# Autodesk Inventor assembly: Shooter Assembly v2 (copy)
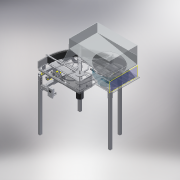
[picture p0: Inventor's stored thumbnail of the model, 180x180]
Saved by Autodesk Inventor 2013 (Build 170138000, 138)
## iProperties
Created: 2013-01-15
Part Number: Shooter Assembly v2 (copy)
Document SubType Name: Assembly
Designer: actoennies
Mass: 9112.82 g
Surface Area: 29351.4 cm^2
Volume: 4689.84 cm^3
Density: 1.9431 g/cm^3
Author: actoennies
## Documents named in this file (49)
- C:\Users\Arpan\Documents\GitHub\frc2013CAD\Launcher\Shooter\Shooter Assembly v2 (copy).iam
- C:\Users\Arpan\Documents\GitHub\frc2013CAD\Launcher\Shooter\Bearing Mount v1.ipt
- C:\Users\Arpan\Documents\GitHub\frc2013CAD\Launcher\Shooter\Outer Rail v1.ipt
- C:\Users\Arpan\Documents\GitHub\frc2013CAD\Launcher\Shooter\Runner Rails v2.ipt
- C:\Users\Arpan\Documents\GitHub\frc2013CAD\Launcher\Shooter\Bearing.ipt
- C:\Users\Arpan\Documents\GitHub\frc2013CAD\Launcher\Shooter\Shooter Mounter.ipt
- C:\Users\Arpan\Documents\GitHub\frc2013CAD\Launcher\Shooter\Bearing Mount 2 v1.ipt
- C:\Users\Arpan\Documents\GitHub\frc2013CAD\Launcher\Shooter\Shorter Shaft.ipt
- C:\Users\Arpan\Documents\GitHub\frc2013CAD\Launcher\Shooter\Spacer Rube.ipt
- C:\Users\Arpan\Documents\GitHub\frc2013CAD\Launcher\Shooter\Edge Mount.ipt
- C:\Users\Arpan\Documents\GitHub\frc2013CAD\Launcher\Shooter\Square Tube.ipt
- C:\Users\Arpan\Documents\GitHub\frc2013CAD\Launcher\Shooter\Flange Bearing Mount Tower.ipt
- C:\Users\Arpan\Documents\GitHub\frc2013CAD\Launcher\Shooter\Flange Bearing Mount Tower Mirror.ipt
- C:\Users\Arpan\Documents\GitHub\frc2013CAD\Launcher\Shooter\Bearing Mount Top.ipt
- C:\Users\Arpan\Documents\GitHub\frc2013CAD\Launcher\Shooter\Square Motor Mount.ipt
- C:\Users\Arpan\Documents\GitHub\frc2013CAD\Launcher\Shooter\Shooter Assembly v2\Design Accelerator\Spur Gears1.iam
- C:\Users\Arpan\Documents\GitHub\frc2013CAD\Launcher\Parts\Imported Components\Snow Blower Motor\Snow Blower Motor.iam
- C:\Users\Arpan\Documents\GitHub\frc2013CAD\Launcher\Shooter\Snowblower Motor Mount.ipt
- C:\Users\Arpan\Documents\GitHub\frc2013CAD\Launcher\Shooter\8mm shaft.ipt
- C:\Users\Arpan\Documents\GitHub\frc2013CAD\Launcher\Shooter\CIM Bearing.ipt
- C:\Users\Arpan\Documents\GitHub\frc2013CAD\Launcher\Shooter\Square Tube 2.ipt
- C:\Users\Arpan\Documents\GitHub\frc2013CAD\Launcher\Parts\CIM Motor\Motors_FR801-001.iam
- C:\Users\Arpan\Documents\GitHub\frc2013CAD\Launcher\Shooter\Cim Mount.ipt
- C:\Users\Arpan\Documents\GitHub\frc2013CAD\Launcher\Shooter\Camera Traffic Light Mount.ipt
- C:\Users\Arpan\Documents\GitHub\frc2013CAD\Launcher\Shooter\Square Tube 3.ipt
- C:\Users\Arpan\Documents\GitHub\frc2013CAD\Launcher\Shooter\edge mount shortened.ipt
- C:\Users\Arpan\Documents\GitHub\frc2013CAD\Launcher\Shooter\Camera.ipt
- C:\Users\Arpan\Documents\GitHub\frc2013CAD\Launcher\Shooter\Square Tube 6.ipt
- C:\Users\Arpan\Documents\GitHub\frc2013CAD\Launcher\Parts\NR-025_5-D(F,D-770).iam
- C:\Users\Arpan\Documents\GitHub\frc2013CAD\Launcher\Parts\Imported Components\E3-X-315-X-D-3-X\E3-X-315-X-D-3-X.ipt
- C:\Users\Arpan\Documents\GitHub\frc2013CAD\Launcher\Shooter\Gusset.ipt
- C:\Users\Arpan\Documents\GitHub\frc2013CAD\Launcher\Shooter\Gusset 2.ipt
- C:\Users\Arpan\Documents\GitHub\frc2013CAD\Launcher\Shooter\Gusset 3.ipt
- C:\Users\Arpan\Documents\GitHub\frc2013CAD\Launcher\Shooter\Gusset 4.ipt
- C:\Users\Arpan\Documents\GitHub\frc2013CAD\Launcher\Shooter\Inner Mount.ipt
- C:\Users\Arpan\Documents\GitHub\frc2013CAD\Launcher\Shooter\Gusset 5.ipt
- C:\Users\Arpan\Documents\GitHub\frc2013CAD\Launcher\Shooter\Hard Stop.ipt
- C:\Users\Arpan\Documents\GitHub\frc2013CAD\Launcher\Shooter\Gusset Connector 2.ipt
- C:\Users\Arpan\Documents\GitHub\frc2013CAD\Launcher\Shooter\L-Channel Strenght.ipt
- C:\Users\Arpan\Documents\GitHub\frc2013CAD\Launcher\Shooter\Gear for Angle.ipt
- C:\Users\Arpan\Documents\GitHub\frc2013CAD\Launcher\Shooter\Encoder Mount 2.ipt
- \\NNHSSRV2.hs.sd203.org\ACToennies$\Robotics\Shooter\Gear Plate.ipt
- \\NNHSSRV2.hs.sd203.org\ACToennies$\Robotics\Shooter\Gear Plate 2.ipt
- C:\Users\Arpan\Documents\GitHub\frc2013CAD\Launcher\Shooter\Wheel Shields.ipt
- C:\Users\Arpan\Documents\GitHub\frc2013CAD\Launcher\Shooter\Rubber Cushion.ipt
- \\NNHSSRV2.hs.sd203.org\ACToennies$\Inventor\Pneumatic Wheel.iam
- C:\Users\Arpan\Documents\GitHub\frc2013CAD\Launcher\Shooter\Puller Hook.ipt
- C:\Users\Arpan\Documents\GitHub\frc2013CAD\Launcher\Shooter\Bucketr.ipt
- C:\Users\Arpan\Documents\GitHub\frc2013CAD\Launcher\Shooter\Hopper.ipt
## Components (71 placed, 48 different names)
1. Bearing Mount v1:1 — Insert:13, Insert:26, Insert:27, Mate:62, Mate:63, Flush:70, Insert:60, Insert:61, Mate:167, Flush:128, Mate:255
2. Outer Rail v1:1 — Insert:13, Insert:48, Flush:70, Mate:252
3. Runner Rails v2:1 — Insert:60, Insert:61, Angle:16, Mate:257, Mate:258, Mate:259, Flush:130, Flush:131
4. Shooter Mounter:1 — Insert:26, Insert:27, Insert:34, Flush:11, Insert:35, Insert:36, Insert:37, Insert:38, Flush:19, Mate:45, Flush:40, Flush:64, Angle:6, Angle:8, Mate:226, Flush:114, Flush:115, Mate:229, Mate:230, Flush:116, Mate:232, Flush:117, Mate:238, Mate:246, Angle:15, Mate:247, Mate:248, Mate:249, Flush:124
5. Spacer Rube:1 — Insert:34, Flush:11
6. Bearing Mount 2 v1:1 — Insert:37, Insert:38, Insert:40
7. Bearing Mount 2 v1:2 — Insert:35, Insert:36, Insert:39
8. Bearing:3 — Insert:40, Flush:13, Mate:14, Mate:15
9. Bearing:4 — Insert:39, Mate:36, Mate:44
10. Shorter Shaft:2 — Flush:13, Mate:14, Mate:15, Mate:38
11. Edge Mount:2 — Flush:34, Mate:104, Flush:48, Mate:106, Flush:68, Mate:174, Flush:74, Mate:220, Mate:222
12. Square Tube:2 — Flush:19, Flush:23, Mate:52, Flush:27, Mate:81, Flush:32, Mate:125, Mate:126, Mate:130, Flush:50, Angle:8, Mate:192, Flush:83, Mate:217, Flush:103, Flush:112, Insert:71, Insert:72
13. Flange Bearing Mount Tower:1 — Insert:43, Flush:112, Flush:113
14. Bearing:5 — Insert:43, Mate:36
15. Flange Bearing Mount Tower Mirror:1 — Flush:55, Mate:135, Flush:111, Insert:70
16. Bearing:6 — Mate:38, Insert:70
17. Bearing Mount Top:1 — Insert:48, Mate:65, Mate:66, Mate:253, Tangent:1
18. Square Motor Mount:1 — Flush:23, Mate:47, Mate:51, Flush:27, Mate:131, Mate:197, Mate:198, Flush:86, Flush:96, Flush:106
19. Spur Gears:1 [sub-assembly] — Mate:44, Mate:45, Flush:25, Mate:46, Angle:2, Flush:64, Angle:6, Mate:227, Mate:228, Mate:231, Mate:233, Flush:120, Mate:239, Flush:122
20. Snow Blower Motor:1 [sub-assembly] — Flush:25, Mate:46, Angle:2, Insert:81, Insert:82, Mate:245
21. Snowblower Motor Mount:1 — Mate:47, Mate:51, Mate:52, Mate:240, Insert:76, Insert:78, Insert:79, Insert:81, Insert:82, Mate:241, Mate:242, Mate:243, Mate:244
22. 8mm shaft:1 — Mate:67, Mate:82, Mate:83, Mate:84, Mate:86, Mate:167, Mate:254
23. CIM Bearing:1 — Mate:65, Mate:66, Mate:67
24. CIM Bearing:2 — Mate:62, Mate:63
25. Square Tube 2:1 — Mate:81, Flush:32, Flush:34, Mate:106, Mate:124, Flush:49, Mate:126, Mate:173, Mate:186, Flush:80, Mate:193, Mate:216, Mate:219, Flush:104, Flush:111, Flush:113
26. Motors_FR801-001:1 [sub-assembly] — Mate:82, Mate:83, Mate:84, Mate:143, Mate:144, Mate:145
27. Cim Mount:1 — Flush:40, Mate:143, Mate:144, Mate:145
28. Camera Traffic Light Mount:1 — Mate:127, Mate:128, Mate:129, Insert:83, Insert:84
29. Square Tube 3:1 — Mate:104, Flush:48, Flush:55, Mate:135, Mate:173, Mate:174, Flush:74, Mate:175, Mate:187, Mate:206, Flush:90, Mate:221, Flush:105, Flush:110
30. edge mount shortened:1 — Mate:124, Mate:125, Flush:49, Mate:196, Flush:85, Mate:215, Flush:102, Mate:218, Mate:223, Flush:107
31. Camera:1 — Mate:127, Mate:128, Mate:129
32. Edge Mount:3 — Mate:130, Mate:131, Flush:50, Mate:199, Mate:209, Flush:97, Mate:212, Mate:260, Mate:261
33. Square Tube 6:1 — Mate:175, Flush:91, Mate:207, Flush:93, Mate:208, Flush:94, Flush:95, Flush:110, Mate:224, Insert:73, Insert:74
34. NR-025_5-D(F,D-770):1 [sub-assembly] — Mate:246, Angle:15, Mate:247, Mate:256, Flush:129
35. Gusset:3 — Mate:186, Flush:80, Mate:187
36. Gusset:4 — Mate:196, Mate:197, Flush:85
37. Gusset:5 — Mate:192, Mate:193, Flush:83
38. Gusset:8 — Mate:198, Mate:199, Flush:86
39. Gusset 2:1 — Mate:206, Flush:90, Flush:91
40. Gusset 3:2 — Mate:209, Flush:96, Flush:97
41. Gusset 3:3 — Mate:208, Flush:94, Flush:95, Flush:108
42. Gusset 3:4 — Mate:207, Flush:93, Mate:225
43. Gusset 4:1 — Mate:212, Mate:260, Mate:261, Insert:83, Insert:84
44. Gusset 4:2
45. Gusset 4:3 — Mate:217, Mate:218, Flush:103
46. Gusset 4:4 — Mate:215, Flush:102, Mate:216
47. Gusset 4:5 — Mate:219, Mate:220, Flush:104
48. Gusset 4:6 — Mate:221, Mate:222, Flush:105
49. Gusset 3:5 — Mate:223, Flush:106, Flush:107
50. Inner Mount:1 — Flush:108, Mate:224, Mate:225
51. Gusset 5:1 — Flush:115, Mate:228, Mate:229
52. Gusset 5:2 — Mate:226, Mate:227, Flush:114
53. Gusset 5:3 — Mate:230, Mate:231, Flush:116
54. Gusset 5:4 — Mate:232, Mate:233, Flush:117
55. Hard Stop:1 — Insert:71, Insert:72
56. Gusset Connector 2:1 — Insert:73, Insert:74
57. L-Channel Strenght:1 — Mate:238, Mate:248, Mate:249, Mate:250, Flush:125
58. Gear for Angle:1 — Flush:120, Mate:239, Mate:240, Flush:121
59. CIM Bearing:3 — Insert:76, Insert:77
60. 8mm shaft:2 — Insert:77, Flush:121
61. E3-X-315-X-D-3-X:2 — Insert:80, Angle:14
62. Encoder Mount 2:1 — Insert:78, Insert:79, Insert:80, Angle:14
63. Gear Plate:1 — Mate:241, Mate:242, Flush:122, Flush:123
64. Gear Plate 2:1 — Mate:243, Mate:244, Flush:123
65. Wheel Shields:1 — Mate:250, Flush:124, Flush:125, Mate:251, Flush:126, Flush:127
66. Wheel Shields:2 — Mate:251, Flush:126, Flush:127, Angle:17
67. Rubber Cushion:1 — Mate:252, Mate:253, Flush:128
68. Pneumatic Wheel:1 [sub-assembly] — Mate:254, Mate:255
69. Puller Hook:1 — Mate:256, Flush:129, Angle:16
70. Bucketr:1 — Mate:257, Tangent:1, Mate:258, Angle:17
71. Hopper:1 — Mate:259, Flush:130, Flush:131
## Relationships (185: Mate 94, Flush 55, Insert 28, Angle 7, Tangent 1)
- Insert:13: Bearing Mount v1:1 ↔ Outer Rail v1:1
- Insert:26: Bearing Mount v1:1 ↔ Shooter Mounter:1
- Insert:27: Bearing Mount v1:1 ↔ Shooter Mounter:1
- Insert:34: Shooter Mounter:1 ↔ Spacer Rube:1
- Flush:11: Shooter Mounter:1 ↔ Spacer Rube:1
- Insert:35: Shooter Mounter:1 ↔ Bearing Mount 2 v1:2
- Insert:36: Shooter Mounter:1 ↔ Bearing Mount 2 v1:2
- Insert:37: Shooter Mounter:1 ↔ Bearing Mount 2 v1:1
- Insert:38: Shooter Mounter:1 ↔ Bearing Mount 2 v1:1
- Insert:39: Bearing Mount 2 v1:2 ↔ Bearing:4
- Insert:40: Bearing Mount 2 v1:1 ↔ Bearing:3
- Flush:13 (-25.4 mm): Bearing:3 ↔ Shorter Shaft:2
- Mate:14: Bearing:3 ↔ Shorter Shaft:2
- Mate:15: Bearing:3 ↔ Shorter Shaft:2
- Insert:43: Flange Bearing Mount Tower:1 ↔ Bearing:5
- Flush:19: Shooter Mounter:1 ↔ Square Tube:2
- Mate:36: Bearing:4 ↔ Bearing:5
- Mate:38: Shorter Shaft:2 ↔ Bearing:6
- Insert:48 (12.7 mm): Outer Rail v1:1 ↔ Bearing Mount Top:1
- Flush:23 (152.4 mm): Square Tube:2 ↔ Square Motor Mount:1
- Mate:44: Bearing:4 ↔ Spur Gears:1
- Mate:45 (25.4 mm): Shooter Mounter:1 ↔ Spur Gears:1
- Flush:25 (-3.175 mm): Spur Gears:1 ↔ Snow Blower Motor:1
- Mate:46: Spur Gears:1 ↔ Snow Blower Motor:1
- Angle:2 (0 deg): Spur Gears:1 ↔ Snow Blower Motor:1
- Mate:47: Square Motor Mount:1 ↔ Snowblower Motor Mount:1
- Mate:51: Square Motor Mount:1 ↔ Snowblower Motor Mount:1
- Mate:52: Square Tube:2 ↔ Snowblower Motor Mount:1
- Flush:27: Square Tube:2 ↔ Square Motor Mount:1
- Mate:62: Bearing Mount v1:1 ↔ CIM Bearing:2
- Mate:63: Bearing Mount v1:1 ↔ CIM Bearing:2
- Mate:65: Bearing Mount Top:1 ↔ CIM Bearing:1
- Mate:66: Bearing Mount Top:1 ↔ CIM Bearing:1
- Mate:67: 8mm shaft:1 ↔ CIM Bearing:1
- Mate:81: Square Tube:2 ↔ Square Tube 2:1
- Flush:32: Square Tube:2 ↔ Square Tube 2:1
- Flush:34: Edge Mount:2 ↔ Square Tube 2:1
- Mate:82: 8mm shaft:1 ↔ Motors_FR801-001:1
- Mate:83: 8mm shaft:1 ↔ Motors_FR801-001:1
- Mate:84: 8mm shaft:1 ↔ Motors_FR801-001:1
- Mate:86: 8mm shaft:1
- Flush:40: Shooter Mounter:1 ↔ Cim Mount:1
- Mate:104: Edge Mount:2 ↔ Square Tube 3:1
- Flush:48: Edge Mount:2 ↔ Square Tube 3:1
- Mate:106: Edge Mount:2 ↔ Square Tube 2:1
- Mate:124: Square Tube 2:1 ↔ edge mount shortened:1
- Mate:125: Square Tube:2 ↔ edge mount shortened:1
- Flush:49: Square Tube 2:1 ↔ edge mount shortened:1
- Mate:126: Square Tube:2 ↔ Square Tube 2:1
- Mate:127: Camera Traffic Light Mount:1 ↔ Camera:1
- Mate:128: Camera Traffic Light Mount:1 ↔ Camera:1
- Mate:129: Camera Traffic Light Mount:1 ↔ Camera:1
- Mate:130: Square Tube:2 ↔ Edge Mount:3
- Mate:131: Square Motor Mount:1 ↔ Edge Mount:3
- Flush:50: Square Tube:2 ↔ Edge Mount:3
- Flush:55: Flange Bearing Mount Tower Mirror:1 ↔ Square Tube 3:1
- Mate:135: Flange Bearing Mount Tower Mirror:1 ↔ Square Tube 3:1
- Mate:143: Motors_FR801-001:1 ↔ Cim Mount:1
- Mate:144: Motors_FR801-001:1 ↔ Cim Mount:1
- Mate:145: Motors_FR801-001:1 ↔ Cim Mount:1
- Flush:64 (3.175 mm): Shooter Mounter:1 ↔ Spur Gears:1
- Flush:68 (-950.9125 mm): Edge Mount:2
- Flush:70: Bearing Mount v1:1 ↔ Outer Rail v1:1
- Insert:60: Bearing Mount v1:1 ↔ Runner Rails v2:1
- Insert:61: Bearing Mount v1:1 ↔ Runner Rails v2:1
- Angle:6 (180 deg): Shooter Mounter:1 ↔ Spur Gears:1
- Mate:167: Bearing Mount v1:1 ↔ 8mm shaft:1
- Angle:8 (180 deg): Shooter Mounter:1 ↔ Square Tube:2
- Mate:173: Square Tube 2:1 ↔ Square Tube 3:1
- Mate:174: Edge Mount:2 ↔ Square Tube 3:1
- Flush:74: Edge Mount:2 ↔ Square Tube 3:1
- Mate:175: Square Tube 3:1 ↔ Square Tube 6:1
- Mate:186: Square Tube 2:1 ↔ Gusset:3
- Flush:80: Square Tube 2:1 ↔ Gusset:3
- Mate:187: Square Tube 3:1 ↔ Gusset:3
- Mate:192: Square Tube:2 ↔ Gusset:5
- Mate:193: Square Tube 2:1 ↔ Gusset:5
- Flush:83: Square Tube:2 ↔ Gusset:5
- Mate:196: edge mount shortened:1 ↔ Gusset:4
- Mate:197: Square Motor Mount:1 ↔ Gusset:4
- Flush:85: edge mount shortened:1 ↔ Gusset:4
- Mate:198: Square Motor Mount:1 ↔ Gusset:8
- Mate:199: Edge Mount:3 ↔ Gusset:8
- Flush:86: Square Motor Mount:1 ↔ Gusset:8
- Mate:206: Square Tube 3:1 ↔ Gusset 2:1
- Flush:90: Square Tube 3:1 ↔ Gusset 2:1
- Flush:91: Square Tube 6:1 ↔ Gusset 2:1
- Mate:207: Square Tube 6:1 ↔ Gusset 3:4
- Flush:93: Square Tube 6:1 ↔ Gusset 3:4
- Mate:208: Square Tube 6:1 ↔ Gusset 3:3
- Flush:94: Square Tube 6:1 ↔ Gusset 3:3
- Flush:95: Square Tube 6:1 ↔ Gusset 3:3
- Mate:209: Edge Mount:3 ↔ Gusset 3:2
- Flush:96: Square Motor Mount:1 ↔ Gusset 3:2
- Flush:97: Edge Mount:3 ↔ Gusset 3:2
- Mate:212: Edge Mount:3 ↔ Gusset 4:1
- Mate:215: edge mount shortened:1 ↔ Gusset 4:4
- Flush:102: edge mount shortened:1 ↔ Gusset 4:4
- Mate:216: Square Tube 2:1 ↔ Gusset 4:4
- Mate:217: Square Tube:2 ↔ Gusset 4:3
- Mate:218: edge mount shortened:1 ↔ Gusset 4:3
- Flush:103: Square Tube:2 ↔ Gusset 4:3
- Mate:219: Square Tube 2:1 ↔ Gusset 4:5
- Mate:220: Edge Mount:2 ↔ Gusset 4:5
- Flush:104: Square Tube 2:1 ↔ Gusset 4:5
- Mate:221: Square Tube 3:1 ↔ Gusset 4:6
- Mate:222: Edge Mount:2 ↔ Gusset 4:6
- Flush:105: Square Tube 3:1 ↔ Gusset 4:6
- Mate:223: edge mount shortened:1 ↔ Gusset 3:5
- Flush:106: Square Motor Mount:1 ↔ Gusset 3:5
- Flush:107: edge mount shortened:1 ↔ Gusset 3:5
- Flush:108: Gusset 3:3 ↔ Inner Mount:1
- Flush:110: Square Tube 3:1 ↔ Square Tube 6:1
- Mate:224: Square Tube 6:1 ↔ Inner Mount:1
- Mate:225: Gusset 3:4 ↔ Inner Mount:1
- Flush:111: Flange Bearing Mount Tower Mirror:1 ↔ Square Tube 2:1
- Flush:112: Square Tube:2 ↔ Flange Bearing Mount Tower:1
- Flush:113: Flange Bearing Mount Tower:1 ↔ Square Tube 2:1
- Insert:70: Flange Bearing Mount Tower Mirror:1 ↔ Bearing:6
- Mate:226: Shooter Mounter:1 ↔ Gusset 5:2
- Mate:227: Spur Gears:1 ↔ Gusset 5:2
- Flush:114: Shooter Mounter:1 ↔ Gusset 5:2
- Flush:115: Shooter Mounter:1 ↔ Gusset 5:1
- Mate:228: Spur Gears:1 ↔ Gusset 5:1
- Mate:229: Shooter Mounter:1 ↔ Gusset 5:1
- Mate:230: Shooter Mounter:1 ↔ Gusset 5:3
- Mate:231: Spur Gears:1 ↔ Gusset 5:3
- Flush:116: Shooter Mounter:1 ↔ Gusset 5:3
- Mate:232: Shooter Mounter:1 ↔ Gusset 5:4
- Mate:233: Spur Gears:1 ↔ Gusset 5:4
- Flush:117: Shooter Mounter:1 ↔ Gusset 5:4
- Insert:71: Square Tube:2 ↔ Hard Stop:1
- Insert:72: Square Tube:2 ↔ Hard Stop:1
- Insert:73: Square Tube 6:1 ↔ Gusset Connector 2:1
- Insert:74: Square Tube 6:1 ↔ Gusset Connector 2:1
- Mate:238: Shooter Mounter:1 ↔ L-Channel Strenght:1
- Flush:120: Spur Gears:1 ↔ Gear for Angle:1
- Mate:239 (304.8 mm): Spur Gears:1 ↔ Gear for Angle:1
- Mate:240: Snowblower Motor Mount:1 ↔ Gear for Angle:1
- Insert:76: Snowblower Motor Mount:1 ↔ CIM Bearing:3
- Insert:77 (-3.175 mm): CIM Bearing:3 ↔ 8mm shaft:2
- Flush:121: Gear for Angle:1 ↔ 8mm shaft:2
- Insert:78: Snowblower Motor Mount:1 ↔ Encoder Mount 2:1
- Insert:79: Snowblower Motor Mount:1 ↔ Encoder Mount 2:1
- Insert:80: E3-X-315-X-D-3-X:2 ↔ Encoder Mount 2:1
- Angle:14 (180 deg): E3-X-315-X-D-3-X:2 ↔ Encoder Mount 2:1
- Insert:81: Snow Blower Motor:1 ↔ Snowblower Motor Mount:1
- Insert:82: Snow Blower Motor:1 ↔ Snowblower Motor Mount:1
- Mate:241: Snowblower Motor Mount:1 ↔ Gear Plate:1
- Mate:242: Snowblower Motor Mount:1 ↔ Gear Plate:1
- Flush:122 (-4.7625 mm): Spur Gears:1 ↔ Gear Plate:1
- Mate:243: Snowblower Motor Mount:1 ↔ Gear Plate 2:1
- Mate:244: Snowblower Motor Mount:1 ↔ Gear Plate 2:1
- Flush:123: Gear Plate:1 ↔ Gear Plate 2:1
- Mate:245: Snow Blower Motor:1
- Mate:246: Shooter Mounter:1 ↔ NR-025_5-D(F,D-770):1
- Angle:15 (180 deg): Shooter Mounter:1 ↔ NR-025_5-D(F,D-770):1
- Mate:247: Shooter Mounter:1 ↔ NR-025_5-D(F,D-770):1
- Mate:248: Shooter Mounter:1 ↔ L-Channel Strenght:1
- Mate:249: Shooter Mounter:1 ↔ L-Channel Strenght:1
- Mate:250: L-Channel Strenght:1 ↔ Wheel Shields:1
- Flush:124: Shooter Mounter:1 ↔ Wheel Shields:1
- Flush:125: L-Channel Strenght:1 ↔ Wheel Shields:1
- Mate:251: Wheel Shields:1 ↔ Wheel Shields:2
- Flush:126: Wheel Shields:1 ↔ Wheel Shields:2
- Flush:127: Wheel Shields:1 ↔ Wheel Shields:2
- Mate:252: Outer Rail v1:1 ↔ Rubber Cushion:1
- Mate:253 (12.7 mm): Bearing Mount Top:1 ↔ Rubber Cushion:1
- Flush:128 (6.35 mm): Bearing Mount v1:1 ↔ Rubber Cushion:1
- Mate:254: 8mm shaft:1 ↔ Pneumatic Wheel:1
- Mate:255 (12.7 mm): Bearing Mount v1:1 ↔ Pneumatic Wheel:1
- Mate:256: NR-025_5-D(F,D-770):1 ↔ Puller Hook:1
- Flush:129 (6.35 mm): NR-025_5-D(F,D-770):1 ↔ Puller Hook:1
- Angle:16 (180 deg): Runner Rails v2:1 ↔ Puller Hook:1
- Mate:257: Runner Rails v2:1 ↔ Bucketr:1
- Tangent:1: Bearing Mount Top:1 ↔ Bucketr:1
- Mate:258: Runner Rails v2:1 ↔ Bucketr:1
- Angle:17 (0 deg): Wheel Shields:2 ↔ Bucketr:1
- Mate:259: Runner Rails v2:1 ↔ Hopper:1
- Flush:130 (25.4 mm): Runner Rails v2:1 ↔ Hopper:1
- Flush:131: Runner Rails v2:1 ↔ Hopper:1
- Mate:260: Edge Mount:3 ↔ Gusset 4:1
- Mate:261: Edge Mount:3 ↔ Gusset 4:1
- Insert:83: Camera Traffic Light Mount:1 ↔ Gusset 4:1
- Insert:84: Camera Traffic Light Mount:1 ↔ Gusset 4:1
